# Autodesk Inventor assembly: ControllerClamp
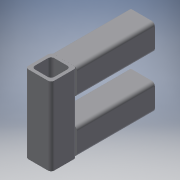
[picture p0: Inventor's stored thumbnail of the model, 180x180]
Saved by Autodesk Inventor 2016 (Build 200138000, 138)
## iProperties
Created: 2016-07-18
Part Number: ControllerClamp
Document SubType Name: Assembly
Designer: cutrones
Author: cutrones
## Documents named in this file (3)
- C:\Users\cutrones\Desktop\motionbase\CAD\MotionBaseCAD\ControllerMount\ControllerClamp.iam
- C:\Users\cutrones\Desktop\motionbase\CAD\MotionBaseCAD\ControllerMount\ClampSide.ipt
- C:\Users\cutrones\Desktop\motionbase\CAD\MotionBaseCAD\ControllerMount\ClampTo.ipt
## Components (3 placed, 2 different names)
1. ClampSide:1 — Mate:1, Flush:1, Flush:2
2. ClampSide:2 — Flush:3, Mate:2, Flush:4
3. ClampTo:1 — Mate:1, Flush:1, Flush:2, Flush:3, Mate:2, Flush:4
## Relationships (6: Flush 4, Mate 2)
- Mate:1: ClampSide:1 ↔ ClampTo:1
- Flush:1: ClampSide:1 ↔ ClampTo:1
- Flush:2: ClampSide:1 ↔ ClampTo:1
- Flush:3: ClampSide:2 ↔ ClampTo:1
- Mate:2: ClampSide:2 ↔ ClampTo:1
- Flush:4: ClampSide:2 ↔ ClampTo:1
